# Autodesk Inventor assembly: Assembly1
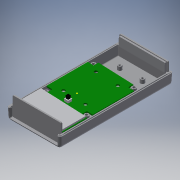
[picture p0: Inventor's stored thumbnail of the model, 180x180]
Saved by Autodesk Inventor 2016 (Build 200138000, 138)
## iProperties
Created: 2015-05-13
Part Number: Assembly1
Document SubType Name: Assembly
Designer: David
Author: David
## Documents named in this file (5)
- C:\Users\David\Documents\GitHub\protochip\casing\Assembly1.iam
- C:\Users\David\Documents\GitHub\protochip\casing\1593X BOTTOM.ipt
- C:\Users\David\Documents\GitHub\protochip\casing\1593X Contoured Endplate.ipt
- C:\Users\David\Documents\GitHub\protochip\casing\1593X Endplate.ipt
- C:\Users\David\Documents\GitHub\protochip\casing\Cheapstat.ipt
## Components (4 placed, 4 different names)
1. 1593X BOTTOM:2 — Mate:1, Mate:2, Mate:3, Mate:4
2. 1593X Contoured Endplate:1 — Mate:1, Mate:2
3. 1593X Endplate:1 — Mate:3, Mate:4, Mate:5
4. Cheapstat:3 — Mate:5
## Relationships (5: Mate 5)
- Mate:1: 1593X BOTTOM:2 ↔ 1593X Contoured Endplate:1
- Mate:2: 1593X BOTTOM:2 ↔ 1593X Contoured Endplate:1
- Mate:3: 1593X BOTTOM:2 ↔ 1593X Endplate:1
- Mate:4: 1593X BOTTOM:2 ↔ 1593X Endplate:1
- Mate:5: 1593X Endplate:1 ↔ Cheapstat:3
